# Autodesk Inventor assembly: RightSideEBoard
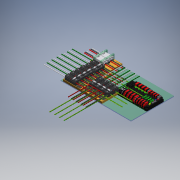
[picture p0: Inventor's stored thumbnail of the model, 180x180]
Saved by Autodesk Inventor 2019 (Build 230136000, 136)
## iProperties
Created: 2020-01-24
Part Number: RightSideEBoard
Document SubType Name: Assembly
Designer: james
Author: james
## Documents named in this file (5)
- F:\JimsRobot\FIRSTRobots\Design\JimsCHS2020FRC\RightSideEBoard.iam
- F:\JimsRobot\FIRSTRobots\Design\JimsCHS2020FRC\SideEBoard.ipt
- F:\JimsRobot\FIRSTRobots\Design\Library\CTR\PDP_CAD\PDP_CAD_REV_1.0\3D\PDP_rev_1.0.ipt
- F:\JimsRobot\FIRSTRobots\Design\Library\Jims\TwoSparkMaxPlate.iam
- F:\JimsRobot\FIRSTRobots\Design\Library\Jims\TwoTalonPlate.iam
## Components (8 placed, 4 different names)
1. SideEBoard:1 — Mate:1, Mate:2, Mate:3, Mate:4, Mate:5, Mate:6, Flush:1, Flush:2, Flush:4, Mate:10, Mate:11
2. PDP_rev_1.0:1 — Mate:1, Mate:10
3. TwoSparkMaxPlate:1 [sub-assembly] — Mate:2, Flush:1, Flush:2, Mate:7
4. TwoTalonPlate:1 [sub-assembly] — Mate:6, Flush:4, Mate:9, Flush:5
5. TwoTalonPlate:2 [sub-assembly] — Mate:5, Mate:8, Mate:12
6. TwoTalonPlate:3 [sub-assembly] — Mate:4, Mate:9, Flush:5
7. TwoTalonPlate:4 [sub-assembly] — Mate:3, Mate:7, Mate:8
8. TwoTalonPlate:5 [sub-assembly] — Mate:11, Mate:12
## Relationships (16: Mate 12, Flush 4)
- Mate:1: SideEBoard:1 ↔ PDP_rev_1.0:1
- Mate:2: SideEBoard:1 ↔ TwoSparkMaxPlate:1
- Mate:3: SideEBoard:1 ↔ TwoTalonPlate:4
- Mate:4: SideEBoard:1 ↔ TwoTalonPlate:3
- Mate:5: SideEBoard:1 ↔ TwoTalonPlate:2
- Mate:6: SideEBoard:1 ↔ TwoTalonPlate:1
- Flush:1: SideEBoard:1 ↔ TwoSparkMaxPlate:1
- Flush:2: SideEBoard:1 ↔ TwoSparkMaxPlate:1
- Mate:7: TwoSparkMaxPlate:1 ↔ TwoTalonPlate:4
- Mate:8: TwoTalonPlate:2 ↔ TwoTalonPlate:4
- Flush:4: SideEBoard:1 ↔ TwoTalonPlate:1
- Mate:9: TwoTalonPlate:1 ↔ TwoTalonPlate:3
- Flush:5: TwoTalonPlate:1 ↔ TwoTalonPlate:3
- Mate:10: SideEBoard:1 ↔ PDP_rev_1.0:1
- Mate:11: SideEBoard:1 ↔ TwoTalonPlate:5
- Mate:12: TwoTalonPlate:2 ↔ TwoTalonPlate:5
